# Autodesk Inventor assembly: Board Pattern
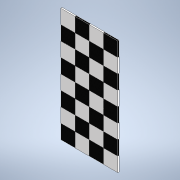
[picture p0: Inventor's stored thumbnail of the model, 180x180]
Saved by Autodesk Inventor 2022 (Build 260153000, 153)
## iProperties
Created: 2022-04-03
Part Number: Board Pattern
Document SubType Name: Assembly
Designer: Nick
Author: Nick
## Documents named in this file (3)
- Y:\Projects\Chess Board\Board Pattern.iam
- Y:\Projects\Chess Board\White Piece.ipt
- Y:\Projects\Chess Board\Black Piece.ipt
## Components (32 placed, 2 different names)
1. White Piece:1
2. Black Piece:1
3. White Piece:9
4. Black Piece:9
5. White Piece:10
6. Black Piece:10
7. White Piece:11
8. Black Piece:11
9. White Piece:12
10. Black Piece:12
11. White Piece:13
12. Black Piece:13
13. White Piece:14
14. Black Piece:14
15. White Piece:15
16. Black Piece:15
17. White Piece:16
18. Black Piece:16
19. White Piece:17
20. Black Piece:17
21. White Piece:18
22. Black Piece:18
23. White Piece:19
24. Black Piece:19
25. White Piece:20
26. Black Piece:20
27. White Piece:21
28. Black Piece:21
29. White Piece:22
30. Black Piece:22
31. White Piece:23
32. Black Piece:23
## Component patterns: (8 elements, first: White Piece:1 + Black Piece:1 + White Piece:9 + Black Piece:9)
## Relationships (9: Flush 5, Mate 4)
- [Mate]: White Piece:1 ↔ Black Piece:1
- [Flush]: White Piece:1 ↔ Black Piece:1
- [Flush]: White Piece:1 ↔ Black Piece:1
- [Flush]: Black Piece:1 ↔ White Piece:9
- [Flush]: Black Piece:1 ↔ White Piece:9
- [Mate]: Black Piece:1 ↔ White Piece:9
- [Flush]: White Piece:1 ↔ Black Piece:9
- [Mate]: White Piece:9 ↔ Black Piece:9
- [Mate]: White Piece:1 ↔ Black Piece:9
## Named parameters: d16_d12 = 0 mm, d18_d14 = 0 mm
